# Autodesk Inventor assembly: Cut Sheet
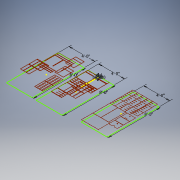
[picture p0: Inventor's stored thumbnail of the model, 180x180]
Saved by Autodesk Inventor 2016 (Build 200138000, 138)
## iProperties
Created: 2017-12-20
Part Number: Cut Sheet
Document SubType Name: Assembly
Designer: mathaetaes
Author: mathaetaes
## Documents named in this file (19)
- E:\Projects\3D Printer\printer projects\My Designs\Bar Cabinet\Cut Sheet.iam
- E:\Projects\3D Printer\printer projects\My Designs\4x8 Plywood.ipt
- E:\Projects\3D Printer\printer projects\My Designs\Bar Cabinet\Base Runner Front.ipt
- E:\Projects\3D Printer\printer projects\My Designs\Bar Cabinet\Base Runner Side.ipt
- E:\Projects\3D Printer\printer projects\My Designs\Bar Cabinet\Top.ipt
- E:\Projects\3D Printer\printer projects\My Designs\Bar Cabinet\Vertical Shelf.ipt
- E:\Projects\3D Printer\printer projects\My Designs\Bar Cabinet\Left Side.ipt
- E:\Projects\3D Printer\printer projects\My Designs\Bar Cabinet\Right Side.ipt
- E:\Projects\3D Printer\printer projects\My Designs\Bar Cabinet\Horizontal Shelf with Lights.ipt
- E:\Projects\3D Printer\printer projects\My Designs\Bar Cabinet\Horizontal Shelf.ipt
- E:\Projects\3D Printer\printer projects\My Designs\Bar Cabinet\Door Side.ipt
- E:\Projects\3D Printer\printer projects\My Designs\Bar Cabinet\Door top.ipt
- E:\Projects\3D Printer\printer projects\My Designs\Bar Cabinet\Door Shelf.ipt
- E:\Projects\3D Printer\printer projects\My Designs\Bar Cabinet\Wine Rack Vertical.ipt
- E:\Projects\3D Printer\printer projects\My Designs\Bar Cabinet\Wine Rack Horizontal.ipt
- E:\Projects\3D Printer\printer projects\My Designs\Bar Cabinet\Back Panel Bottom.ipt
- E:\Projects\3D Printer\printer projects\My Designs\Bar Cabinet\Wine Bottle Rack Back Panel.ipt
- E:\Projects\3D Printer\printer projects\My Designs\Bar Cabinet\Door moulding slide-in panel.ipt
- E:\Projects\3D Printer\printer projects\My Designs\Bar Cabinet\Cabinet Back Sheet.ipt
## Components (47 placed, 18 different names)
1. 4x8 Plywood:1
2. Top:1
3. Base Runner Front:1
4. Base Runner Front:2
5. Base Runner Side:1
6. Base Runner Side:2
7. 4x8 Plywood:2
8. Vertical Shelf:1
9. Left Side:1
10. Right Side:1
11. Horizontal Shelf with Lights:1
12. Horizontal Shelf with Lights:2
13. Horizontal Shelf:1
14. Horizontal Shelf:2
15. Door Side:1
16. Door Side:2
17. Door Side:3
18. Door Side:4
19. Door top:1
20. Door top:2
21. Door top:3
22. Door top:4
23. Door Shelf:1
24. Door Shelf:2
25. Door Shelf:3
26. 4x8 Plywood:3
27. Wine Rack Vertical:1 — Flush:1, Flush:4, Flush:18, Mate:2, Flush:31, Flush:33
28. Wine Rack Vertical:2 — Flush:1, Flush:2, Flush:4, Flush:5
29. Wine Rack Vertical:3 — Flush:2, Flush:3, Flush:5, Flush:6
30. Wine Rack Vertical:4 — Flush:3, Flush:6, Flush:7, Flush:32
31. Wine Rack Vertical:5 — Flush:7, Flush:8, Flush:32
32. Wine Rack Vertical:6 — Flush:17, Flush:18, Flush:24, Flush:40
33. Wine Rack Horizontal:1 — Flush:10, Flush:11, Flush:28, Flush:29
34. Wine Rack Horizontal:2 — Flush:12, Flush:13, Flush:27, Mate:2, Flush:31, Flush:33, Flush:34, Mate:3
35. Wine Rack Horizontal:3 — Flush:11, Flush:12, Flush:27, Flush:28
36. Wine Rack Horizontal:4 — Flush:9, Flush:10, Flush:29, Flush:30
37. Wine Rack Horizontal:5 — Flush:8, Flush:9, Flush:30
38. Wine Rack Horizontal:6 — Flush:13, Flush:14, Flush:34, Flush:35, Flush:37, Mate:3, Mate:4
39. Back Panel Bottom:1 — Flush:19, Flush:22, Flush:24, Flush:25, Mate:1
40. Back Panel Bottom:2 — Flush:20, Flush:23, Flush:26
41. Wine Bottle Rack Back Panel:1 — Flush:19, Flush:20, Flush:25, Flush:26
42. Door moulding slide-in panel:1 — Flush:21, Flush:35, Flush:36, Mate:4, Mate:5
43. Door moulding slide-in panel:2 — Flush:21, Flush:22
44. Wine Rack Horizontal:7 — Flush:14, Flush:15, Flush:37, Flush:38
45. Wine Rack Horizontal:8 — Flush:15, Flush:16, Flush:38, Flush:39
46. Wine Rack Horizontal:9 — Flush:16, Flush:17, Mate:1, Flush:39, Flush:40
47. Cabinet Back Sheet:1 — Flush:23, Flush:36, Mate:5
## Relationships (45: Flush 40, Mate 5)
- Flush:1: Wine Rack Vertical:1 ↔ Wine Rack Vertical:2
- Flush:2: Wine Rack Vertical:2 ↔ Wine Rack Vertical:3
- Flush:3: Wine Rack Vertical:3 ↔ Wine Rack Vertical:4
- Flush:4: Wine Rack Vertical:1 ↔ Wine Rack Vertical:2
- Flush:5: Wine Rack Vertical:2 ↔ Wine Rack Vertical:3
- Flush:6: Wine Rack Vertical:3 ↔ Wine Rack Vertical:4
- Flush:7: Wine Rack Vertical:4 ↔ Wine Rack Vertical:5
- Flush:8: Wine Rack Vertical:5 ↔ Wine Rack Horizontal:5
- Flush:9: Wine Rack Horizontal:4 ↔ Wine Rack Horizontal:5
- Flush:10: Wine Rack Horizontal:1 ↔ Wine Rack Horizontal:4
- Flush:11: Wine Rack Horizontal:1 ↔ Wine Rack Horizontal:3
- Flush:12: Wine Rack Horizontal:2 ↔ Wine Rack Horizontal:3
- Flush:13: Wine Rack Horizontal:2 ↔ Wine Rack Horizontal:6
- Flush:14: Wine Rack Horizontal:6 ↔ Wine Rack Horizontal:7
- Flush:15: Wine Rack Horizontal:7 ↔ Wine Rack Horizontal:8
- Flush:16: Wine Rack Horizontal:8 ↔ Wine Rack Horizontal:9
- Flush:17: Wine Rack Vertical:6 ↔ Wine Rack Horizontal:9
- Flush:18: Wine Rack Vertical:1 ↔ Wine Rack Vertical:6
- Flush:19: Back Panel Bottom:1 ↔ Wine Bottle Rack Back Panel:1
- Flush:20: Back Panel Bottom:2 ↔ Wine Bottle Rack Back Panel:1
- Flush:21: Door moulding slide-in panel:1 ↔ Door moulding slide-in panel:2
- Flush:22: Back Panel Bottom:1 ↔ Door moulding slide-in panel:2
- Flush:23: Back Panel Bottom:2 ↔ Cabinet Back Sheet:1
- Flush:24: Wine Rack Vertical:6 ↔ Back Panel Bottom:1
- Flush:25: Back Panel Bottom:1 ↔ Wine Bottle Rack Back Panel:1
- Flush:26: Back Panel Bottom:2 ↔ Wine Bottle Rack Back Panel:1
- Mate:1 (3.175 mm): Back Panel Bottom:1 ↔ Wine Rack Horizontal:9
- Flush:27: Wine Rack Horizontal:2 ↔ Wine Rack Horizontal:3
- Flush:28: Wine Rack Horizontal:1 ↔ Wine Rack Horizontal:3
- Flush:29: Wine Rack Horizontal:1 ↔ Wine Rack Horizontal:4
- Flush:30: Wine Rack Horizontal:4 ↔ Wine Rack Horizontal:5
- Mate:2 (3.175 mm): Wine Rack Vertical:1 ↔ Wine Rack Horizontal:2
- Flush:31: Wine Rack Vertical:1 ↔ Wine Rack Horizontal:2
- Flush:32: Wine Rack Vertical:4 ↔ Wine Rack Vertical:5
- Flush:33: Wine Rack Vertical:1 ↔ Wine Rack Horizontal:2
- Flush:34: Wine Rack Horizontal:2 ↔ Wine Rack Horizontal:6
- Flush:35: Wine Rack Horizontal:6 ↔ Door moulding slide-in panel:1
- Flush:36: Door moulding slide-in panel:1 ↔ Cabinet Back Sheet:1
- Flush:37: Wine Rack Horizontal:6 ↔ Wine Rack Horizontal:7
- Flush:38: Wine Rack Horizontal:7 ↔ Wine Rack Horizontal:8
- Flush:39: Wine Rack Horizontal:8 ↔ Wine Rack Horizontal:9
- Flush:40: Wine Rack Vertical:6 ↔ Wine Rack Horizontal:9
- Mate:3 (3.175 mm): Wine Rack Horizontal:2 ↔ Wine Rack Horizontal:6
- Mate:4 (3.175 mm): Wine Rack Horizontal:6 ↔ Door moulding slide-in panel:1
- Mate:5 (3.175 mm): Door moulding slide-in panel:1 ↔ Cabinet Back Sheet:1
